# Autodesk Inventor assembly: new metal drivetrain motor mount
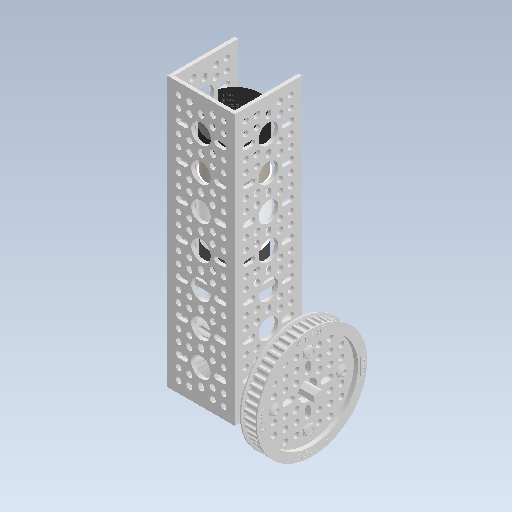
[picture p0: Inventor's stored thumbnail of the model, 512x512]
Saved by Autodesk Inventor 2020 (Build 240168000, 168)
## iProperties
Created: 2020-02-22
Part Number: new metal drivetrain motor mount
Document SubType Name: Assembly
Designer: jackm
Author: jackm
## Documents named in this file (9)
- D:\FTC8863\2019 Robot\Mecanum Drive Train Metal\new metal drivetrain motor mount.iam
- D:\FTC8863\GoBilda\3204 Parts\3204-0002-0001 assembly.ipt
- D:\FTC8863\GoBilda\1702 Parts\1702-0032-0002 assembly.ipt
- D:\FTC8863\Andymark\am-3461a+NeveRest+Orbital+3.7+REV2.ipt
- D:\FTC8863\GoBilda\3204 Parts\1120-0007-0192.ipt
- D:\FTC8863\GoBilda\3415 Parts\3415-0014-0048 Assembly.ipt
- D:\FTC8863\GoBilda\1309 Parts\1309-0016-4008 assembly.ipt
- D:\FTC8863\GoBilda\1309 Parts\2102-0008-0090.ipt
- D:\FTC8863\GoBilda\1601 Parts\1601-0014-0008.ipt
## Components (9 placed, 8 different names)
1. 3204-0002-0001 assembly:1 — Mate:12
2. 1702-0032-0002 assembly:1 — Mate:10, Mate:11, Mate:17, Mate:18, Mate:19
3. am-3461a+NeveRest+Orbital+3.7+REV2:1 — Mate:10, Mate:11, Mate:12
4. 2102-0008-0090:1 — Flush:1, Mate:27
5. 1120-0007-0192:1 — Mate:17, Mate:18, Mate:19, Mate:20, Mate:21, Mate:22, Mate:23, Mate:28
6. 3415-0014-0048 Assembly:1 — Mate:24, Mate:25, Mate:26, Mate:27
7. 1309-0016-4008 assembly:1 — Mate:24, Mate:25, Mate:26, Mate:28
8. 1601-0014-0008:1 — Mate:20, Mate:21, Flush:1
9. 1601-0014-0008:2 — Mate:22, Mate:23
## Relationships (17: Mate 16, Flush 1)
- [Mate]: 3204-0002-0001 assembly:1 ↔ 2102-0008-0090:1
- Mate:10: 1702-0032-0002 assembly:1 ↔ am-3461a+NeveRest+Orbital+3.7+REV2:1
- Mate:11: 1702-0032-0002 assembly:1 ↔ am-3461a+NeveRest+Orbital+3.7+REV2:1
- Mate:12: 3204-0002-0001 assembly:1 ↔ am-3461a+NeveRest+Orbital+3.7+REV2:1
- Mate:17: 1702-0032-0002 assembly:1 ↔ 1120-0007-0192:1
- Mate:18: 1702-0032-0002 assembly:1 ↔ 1120-0007-0192:1
- Mate:19: 1702-0032-0002 assembly:1 ↔ 1120-0007-0192:1
- Mate:20: 1120-0007-0192:1 ↔ 1601-0014-0008:1
- Mate:21: 1120-0007-0192:1 ↔ 1601-0014-0008:1
- Mate:22: 1120-0007-0192:1 ↔ 1601-0014-0008:2
- Mate:23: 1120-0007-0192:1 ↔ 1601-0014-0008:2
- Flush:1 (-5.08 mm): 2102-0008-0090:1 ↔ 1601-0014-0008:1
- Mate:24: 3415-0014-0048 Assembly:1 ↔ 1309-0016-4008 assembly:1
- Mate:25: 3415-0014-0048 Assembly:1 ↔ 1309-0016-4008 assembly:1
- Mate:26: 3415-0014-0048 Assembly:1 ↔ 1309-0016-4008 assembly:1
- Mate:27: 2102-0008-0090:1 ↔ 3415-0014-0048 Assembly:1
- Mate:28 (13.9954 mm): 1120-0007-0192:1 ↔ 1309-0016-4008 assembly:1
